# Autodesk Inventor assembly: Omni Robot v2
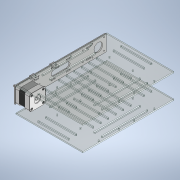
[picture p0: Inventor's stored thumbnail of the model, 180x180]
Saved by Autodesk Inventor 2021 (Build 250183000, 183)
## iProperties
Created: 2022-08-18
Part Number: Omni Robot v2
Document SubType Name: Assembly
Designer: 21155060
Author: 21155060
## Documents named in this file (5)
- C:\Users\21155060\Downloads\Omni-Robot-3D-main\Omni Robot v2.iam
- C:\Users\21155060\Downloads\Omni-Robot-3D-main\Base.ipt
- C:\Users\21155060\Downloads\Omni-Robot-3D-main\Lateral_Acrilico.ipt
- C:\Users\21155060\Downloads\Omni-Robot-3D-main\cantoneira.ipt
- C:\Users\21155060\Downloads\Omni-Robot-3D-main\MINEBEA 05701607 stepper motor.ipt
## Components (6 placed, 4 different names)
1. Base:1 — Alinhado:1, Alinhado:2, Alinhado:3
2. Base:2 — Alinhado:1, Alinhado:2, Coincidente:4, Coincidente:5
3. Lateral_Acrilico:1 — Coincidente:1, Coincidente:2, Coincidente:3, Alinhado:3, Coincidente:6, Coincidente:7, Coincidente:8, Coincidente:9, Alinhado:4, Alinhado:5
4. cantoneira:1 — Coincidente:1, Coincidente:2, Coincidente:3, Coincidente:4, Coincidente:5
5. cantoneira:2 — Coincidente:6, Coincidente:7, Coincidente:8
6. MINEBEA 05701607 stepper motor:1 — Coincidente:9, Alinhado:4, Alinhado:5
## Relationships (14: Mate 9, Flush 5)
- Alinhado:1 [Flush]: Base:1 ↔ Base:2
- Alinhado:2 [Flush]: Base:1 ↔ Base:2
- Coincidente:1 [Mate]: Lateral_Acrilico:1 ↔ cantoneira:1
- Coincidente:2 [Mate]: Lateral_Acrilico:1 ↔ cantoneira:1
- Coincidente:3 [Mate] (0.1 mm): Lateral_Acrilico:1 ↔ cantoneira:1
- Coincidente:4 [Mate]: Base:2 ↔ cantoneira:1
- Coincidente:5 [Mate]: Base:2 ↔ cantoneira:1
- Alinhado:3 [Flush]: Base:1 ↔ Lateral_Acrilico:1
- Coincidente:6 [Mate]: Lateral_Acrilico:1 ↔ cantoneira:2
- Coincidente:7 [Mate] (0.1 mm): Lateral_Acrilico:1 ↔ cantoneira:2
- Coincidente:8 [Mate]: Lateral_Acrilico:1 ↔ cantoneira:2
- Coincidente:9 [Mate]: Lateral_Acrilico:1 ↔ MINEBEA 05701607 stepper motor:1
- Alinhado:4 [Flush]: Lateral_Acrilico:1 ↔ MINEBEA 05701607 stepper motor:1
- Alinhado:5 [Flush]: Lateral_Acrilico:1 ↔ MINEBEA 05701607 stepper motor:1
